# Autodesk Inventor assembly: MG-Color Detect
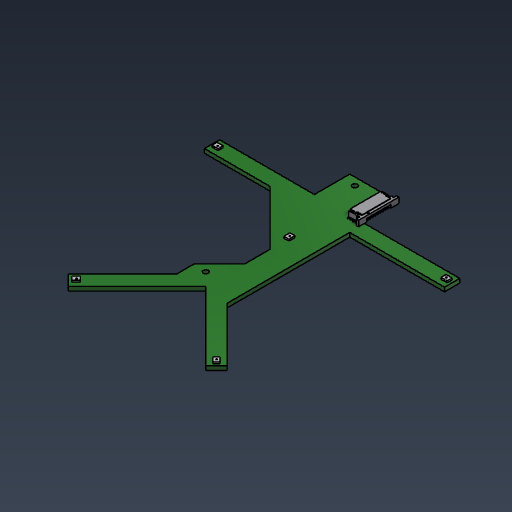
[picture p0: Inventor's stored thumbnail of the model, 512x512]
Saved by Autodesk Inventor 2023.1 (Build 271208000, 208)
## iProperties
Part Number: MG-Color Detect
Material: Generisch
Document SubType Name: Assembly
Designer: rYan
Mass: 4.61652 g
Surface Area: 53.4033 cm^2
Volume: 3.39753 cm^3
Density: 1.35879 g/cm^3
Author: rYan
## Documents named in this file (4)
- D:\TIGERsGIT\Hardware\mechanik\2024\Inventor\Robot\Electronics\MG-Color Detect.iam
- D:\TIGERsGIT\Hardware\mechanik\2024\Inventor\Robot\Electronics\Color Detect PCB.ipt
- D:\TIGERsGIT\Hardware\mechanik\2024\Inventor\Purchased Parts\TE FFC Con 8pin 1mm bottom.ipt
- D:\TIGERsGIT\Hardware\mechanik\2024\Inventor\Purchased Parts\TCS3472.ipt
## Components (7 placed, 3 different names)
1. Color Detect PCB:1 — Fluchtend:1, Fluchtend:2, Fluchtend:3, Passend:1, Fluchtend:5, Passend:2, Passend:3, Passend:4, Passend:5, Passend:6, Fluchtend:6, Fluchtend:7, Fluchtend:8, Fluchtend:9, Fluchtend:10, Fluchtend:11, Fluchtend:12, Fluchtend:13
2. TE FFC Con 8pin 1mm bottom:1 — Passend:1, Fluchtend:4, Fluchtend:5
3. TCS3472:1 — Passend:6, Fluchtend:10, Fluchtend:11
4. TCS3472:2 — Passend:2, Fluchtend:12, Fluchtend:13
5. TCS3472:3 — Passend:4, Fluchtend:8, Fluchtend:9
6. TCS3472:4 — Passend:3, Fluchtend:6, Fluchtend:7
7. TCS3472:5 — Passend:5, Passend:7, Fluchtend:14
## Relationships (21: Flush 14, Mate 7)
- Fluchtend:1 [Flush]: Color Detect PCB:1
- Fluchtend:2 [Flush]: Color Detect PCB:1
- Fluchtend:3 [Flush]: Color Detect PCB:1
- Passend:1 [Mate]: Color Detect PCB:1 ↔ TE FFC Con 8pin 1mm bottom:1
- Fluchtend:4 [Flush] (-36.5 mm): TE FFC Con 8pin 1mm bottom:1
- Fluchtend:5 [Flush]: Color Detect PCB:1 ↔ TE FFC Con 8pin 1mm bottom:1
- Passend:2 [Mate]: Color Detect PCB:1 ↔ TCS3472:2
- Passend:3 [Mate]: Color Detect PCB:1 ↔ TCS3472:4
- Passend:4 [Mate]: Color Detect PCB:1 ↔ TCS3472:3
- Passend:5 [Mate]: Color Detect PCB:1 ↔ TCS3472:5
- Passend:6 [Mate]: Color Detect PCB:1 ↔ TCS3472:1
- Fluchtend:6 [Flush] (1 mm): Color Detect PCB:1 ↔ TCS3472:4
- Fluchtend:7 [Flush] (3 mm): Color Detect PCB:1 ↔ TCS3472:4
- Fluchtend:8 [Flush] (1 mm): Color Detect PCB:1 ↔ TCS3472:3
- Fluchtend:9 [Flush] (2 mm): Color Detect PCB:1 ↔ TCS3472:3
- Fluchtend:10 [Flush] (1 mm): Color Detect PCB:1 ↔ TCS3472:1
- Fluchtend:11 [Flush] (2 mm): Color Detect PCB:1 ↔ TCS3472:1
- Fluchtend:12 [Flush] (1 mm): Color Detect PCB:1 ↔ TCS3472:2
- Fluchtend:13 [Flush] (2 mm): Color Detect PCB:1 ↔ TCS3472:2
- Passend:7 [Mate] (10 mm): TCS3472:5
- Fluchtend:14 [Flush]: TCS3472:5
